# Autodesk Inventor assembly: podest duzy polowka
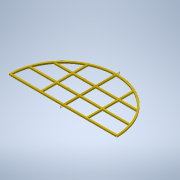
[picture p0: Inventor's stored thumbnail of the model, 180x180]
Saved by Autodesk Inventor 2021 (Build 250183000, 183)
## iProperties
Created: 2024-04-18
Part Number: podest duzy polowka
Document SubType Name: Assembly
Designer: Michal
Author: Michal
## Documents named in this file (12)
- C:\Users\Michal\Documents\GitHub\PNW_PhotoBoothFrame_3D\podest duzy polowka.iam
- C:\Users\Michal\Documents\GitHub\PNW_PhotoBoothFrame_3D\Luk R2000 podest.ipt
- C:\Users\Michal\Documents\GitHub\PNW_PhotoBoothFrame_3D\podest duzy profil 1.ipt
- C:\Users\Michal\Documents\GitHub\PNW_PhotoBoothFrame_3D\podest duzy profil 2.ipt
- C:\Users\Michal\Documents\GitHub\PNW_PhotoBoothFrame_3D\podest duzy profil 3.ipt
- C:\Users\Michal\Documents\GitHub\PNW_PhotoBoothFrame_3D\podest duzy profil 4.ipt
- C:\Users\Michal\Documents\GitHub\PNW_PhotoBoothFrame_3D\podest duzy profil 5.ipt
- C:\Users\Michal\Documents\GitHub\PNW_PhotoBoothFrame_3D\podest duzy profil 6.ipt
- C:\Users\Michal\Documents\GitHub\PNW_PhotoBoothFrame_3D\podest duzy profil 3_MIR.ipt
- C:\Users\Michal\Documents\GitHub\PNW_PhotoBoothFrame_3D\podest duzy profil 4_MIR.ipt
- C:\Users\Michal\Documents\GitHub\PNW_PhotoBoothFrame_3D\podest duzy profil 5_MIR.ipt
- C:\Users\Michal\Documents\GitHub\PNW_PhotoBoothFrame_3D\podest duzy profil 6_MIR.ipt
## Components (13 placed, 11 different names)
1. Luk R2000 podest:1 — Flush:26, Flush:27, Mate:35, Flush:37, Mate:39, Mate:41
2. podest duzy profil 1:1 — Flush:37, Mate:36, Flush:38, Mate:37, Mate:40, Flush:40, Mate:45
3. podest duzy profil 2:1 — Mate:37, Mate:38, Mate:39, Mate:46, Mate:47, Mate:48, Mate:49
4. podest duzy profil 3:1 — Mate:40, Flush:39, Mate:41, Mate:42, Mate:44
5. podest duzy profil 4:1 — Mate:42, Mate:43, Flush:40, Flush:41, Flush:42
6. podest duzy profil 5:1 — Mate:44, Mate:45, Flush:41, Flush:43
7. podest duzy profil 6:1 — Mate:46, Mate:47, Flush:42
8. podest duzy profil 6:2 — Mate:48, Flush:43, Mate:49
9. podest duzy profil 3_MIR:1 — Mate:50, Mate:51, Mate:52
10. podest duzy profil 4_MIR:1 — Flush:44, Mate:51, Flush:45, Flush:46
11. podest duzy profil 5_MIR:1 — Flush:45, Mate:52, Flush:47
12. podest duzy profil 6_MIR:1 — Flush:46
13. podest duzy profil 6_MIR:2 — Flush:47
## Relationships (31: Mate 18, Flush 13)
- Flush:26: Luk R2000 podest:1
- Flush:27: Luk R2000 podest:1
- Mate:35: Luk R2000 podest:1
- Flush:37: Luk R2000 podest:1 ↔ podest duzy profil 1:1
- Mate:36: podest duzy profil 1:1
- Flush:38: podest duzy profil 1:1
- Mate:37: podest duzy profil 1:1 ↔ podest duzy profil 2:1
- Mate:38: podest duzy profil 2:1
- Mate:39: Luk R2000 podest:1 ↔ podest duzy profil 2:1
- Mate:40: podest duzy profil 1:1 ↔ podest duzy profil 3:1
- Flush:39: podest duzy profil 3:1
- Mate:41: Luk R2000 podest:1 ↔ podest duzy profil 3:1
- Mate:42: podest duzy profil 3:1 ↔ podest duzy profil 4:1
- Mate:43: podest duzy profil 4:1
- Flush:40 (300 mm): podest duzy profil 1:1 ↔ podest duzy profil 4:1
- Mate:44: podest duzy profil 3:1 ↔ podest duzy profil 5:1
- Mate:45: podest duzy profil 1:1 ↔ podest duzy profil 5:1
- Flush:41 (300 mm): podest duzy profil 4:1 ↔ podest duzy profil 5:1
- Mate:46: podest duzy profil 2:1 ↔ podest duzy profil 6:1
- Mate:47: podest duzy profil 2:1 ↔ podest duzy profil 6:1
- Flush:42: podest duzy profil 4:1 ↔ podest duzy profil 6:1
- Mate:48: podest duzy profil 2:1 ↔ podest duzy profil 6:2
- Flush:43: podest duzy profil 5:1 ↔ podest duzy profil 6:2
- Mate:49: podest duzy profil 2:1 ↔ podest duzy profil 6:2
- Mate:50: podest duzy profil 3_MIR:1
- Flush:44: podest duzy profil 4_MIR:1
- Mate:51: podest duzy profil 3_MIR:1 ↔ podest duzy profil 4_MIR:1
- Flush:45 (300 mm): podest duzy profil 4_MIR:1 ↔ podest duzy profil 5_MIR:1
- Mate:52: podest duzy profil 3_MIR:1 ↔ podest duzy profil 5_MIR:1
- Flush:46: podest duzy profil 4_MIR:1 ↔ podest duzy profil 6_MIR:1
- Flush:47: podest duzy profil 5_MIR:1 ↔ podest duzy profil 6_MIR:2
